# Autodesk Inventor assembly: Assembly1
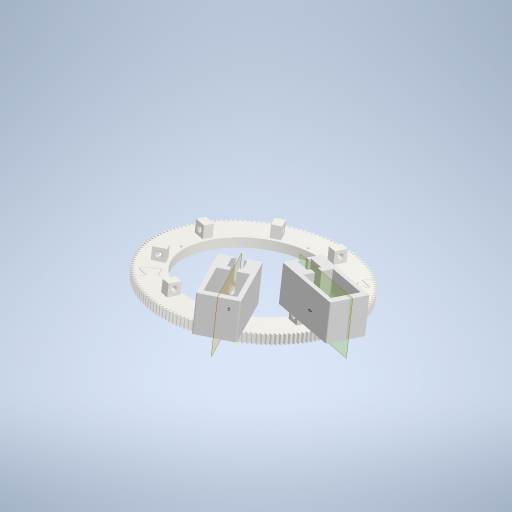
[picture p0: Inventor's stored thumbnail of the model, 512x512]
Saved by Autodesk Inventor 2023 (Build 270158000, 158)
## iProperties
Created: 2023-04-05
Part Number: Assembly1
Document SubType Name: Assembly
Designer: czapa
Author: czapa
## Documents named in this file (3)
- C:\Users\czapa\OneDrive\Documents\GitHub\S.P.I.C.E\3D Models\Version1\stls\Assembly1.iam
- C:\Users\czapa\OneDrive\Documents\GitHub\S.P.I.C.E\3D Models\Version1\BearingGearMk2.ipt
- C:\Users\czapa\OneDrive\Documents\GitHub\S.P.I.C.E\3D Models\housing_V3.ipt
## Components (4 placed, 2 different names)
1. Spur Gear2:1 — Flush:1, Mate:1, Mate:4
2. Spur Gear2:2 — Flush:1, Mate:1, Mate:2, Mate:3, Flush:2, Mate:4, Mate:5, Flush:3, Mate:6
3. housing_V3:1 — Mate:2, Mate:3, Flush:2
4. housing_V3:2 — Mate:5, Flush:3, Mate:6
## Relationships (9: Mate 6, Flush 3)
- Flush:1: Spur Gear2:1 ↔ Spur Gear2:2
- Mate:1: Spur Gear2:1 ↔ Spur Gear2:2
- Mate:2: Spur Gear2:2 ↔ housing_V3:1
- Mate:3: Spur Gear2:2 ↔ housing_V3:1
- Flush:2: Spur Gear2:2 ↔ housing_V3:1
- Mate:4: Spur Gear2:1 ↔ Spur Gear2:2
- Mate:5: Spur Gear2:2 ↔ housing_V3:2
- Flush:3: Spur Gear2:2 ↔ housing_V3:2
- Mate:6: Spur Gear2:2 ↔ housing_V3:2
